# Autodesk Inventor assembly: Ball Bearing, No Insert_CPY
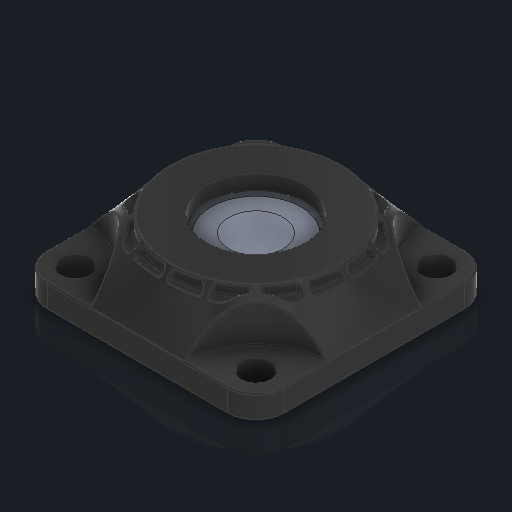
[picture p0: Inventor's stored thumbnail of the model, 512x512]
Saved by Autodesk Inventor 2023.2 (Build 272271030, 271C)
## iProperties
Created: 2022-08-18
Part Number: Ball Bearing, No Insert_CPY
Document SubType Name: Assembly
Designer: Michael
Author: ylu12
## Documents named in this file (3)
- C:\Users\black\OneDrive\Pictures\Documents\VEX CAD\VEX-CAD-Inventor-1.4.0\Motion\Ball Bearing\Ball Bearing, No Insert_CPY.iam
- C:\Users\black\OneDrive\Pictures\Documents\VEX CAD\VEX-CAD-Inventor-1.4.0\Motion\Reference Files\Ball Bearing Housing_CPY.ipt
- C:\Users\black\OneDrive\Pictures\Documents\VEX CAD\VEX-CAD-Inventor-1.4.0\Motion\Reference Files\Ball Bearing_CPY.ipt
## Components (2 placed, 2 different names)
1. Ball Bearing Housing_CPY:1 — Mate:2, Mate:1
2. Ball Bearing_CPY:1 — Mate:2, Mate:1
## Relationships (2: Mate 2)
- Mate:2: Ball Bearing Housing_CPY:1 ↔ Ball Bearing_CPY:1
- Mate:1: Ball Bearing Housing_CPY:1 ↔ Ball Bearing_CPY:1
